# Autodesk Inventor assembly: assembled
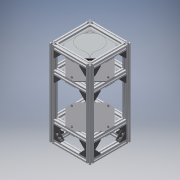
[picture p0: Inventor's stored thumbnail of the model, 180x180]
Saved by Autodesk Inventor 2016 (Build 200138000, 138)
## iProperties
Created: 2016-07-21
Part Number: assembled
Document SubType Name: Assembly
Designer: Jonathan
Author: Jonathan
## Documents named in this file (5)
- C:\Users\Jonathan\Documents\Projects\muonTelescope\assembled.iam
- C:\Users\Jonathan\Documents\Projects\muonTelescope\frame\frame.iam
- C:\Users\Jonathan\Documents\Projects\muonTelescope\frame\separator\assembled cover.iam
- C:\Users\Jonathan\Documents\Projects\muonTelescope\panel assembly\panel assembly.iam
- C:\Users\Jonathan\Documents\Projects\muonTelescope\frameSpecifications.xlsx
## Components (9 placed, 3 different names)
1. frame:1 [sub-assembly] — Mate:1, Mate:2, Mate:3, Flush:5, Flush:6, Mate:8, Mate:9, Flush:15, Flush:16, Angle:1
2. assembled cover:1 [sub-assembly] — Mate:2, Flush:1, Flush:2, Flush:3, Flush:4, Mate:11, Mate:13
3. assembled cover:2 [sub-assembly] — Mate:1, Flush:1, Flush:4, Flush:5, Flush:6, Mate:10
4. assembled cover:3 [sub-assembly] — Mate:3, Flush:2, Flush:3, Mate:12
5. assembled cover:5 [sub-assembly] — Flush:12, Flush:13, Mate:8, Flush:15, Flush:16
6. assembled cover:6 [sub-assembly] — Flush:12, Flush:13, Mate:9
7. panel assembly:1 [sub-assembly] — Flush:20, Mate:10, Flush:23, Flush:24, Angle:1
8. panel assembly:3 [sub-assembly] — Flush:20, Flush:21, Flush:22, Flush:23, Flush:24, Mate:11, Mate:13
9. panel assembly:4 [sub-assembly] — Flush:21, Flush:22, Mate:12
## Relationships (25: Flush 15, Mate 9, Angle 1)
- Mate:1: frame:1 ↔ assembled cover:2
- Mate:2: frame:1 ↔ assembled cover:1
- Mate:3: frame:1 ↔ assembled cover:3
- Flush:1: assembled cover:1 ↔ assembled cover:2
- Flush:2: assembled cover:1 ↔ assembled cover:3
- Flush:3: assembled cover:1 ↔ assembled cover:3
- Flush:4: assembled cover:1 ↔ assembled cover:2
- Flush:5: frame:1 ↔ assembled cover:2
- Flush:6: frame:1 ↔ assembled cover:2
- Flush:12: assembled cover:5 ↔ assembled cover:6
- Flush:13: assembled cover:5 ↔ assembled cover:6
- Mate:8: frame:1 ↔ assembled cover:5
- Mate:9: frame:1 ↔ assembled cover:6
- Flush:15: frame:1 ↔ assembled cover:5
- Flush:16: frame:1 ↔ assembled cover:5
- Flush:20: panel assembly:1 ↔ panel assembly:3
- Flush:21: panel assembly:3 ↔ panel assembly:4
- Flush:22: panel assembly:3 ↔ panel assembly:4
- Mate:10: assembled cover:2 ↔ panel assembly:1
- Flush:23: panel assembly:1 ↔ panel assembly:3
- Flush:24: panel assembly:1 ↔ panel assembly:3
- Angle:1 (0 deg): frame:1 ↔ panel assembly:1
- Mate:11: assembled cover:1 ↔ panel assembly:3
- Mate:12: assembled cover:3 ↔ panel assembly:4
- Mate:13: assembled cover:1 ↔ panel assembly:3
## Named parameters: height = 400 mm, width = 150 mm, topSeparation = 100 mm, botSeparation = 200 mm, panelChamfer = 75 mm
